# Autodesk Inventor assembly: 回転軸フレーム
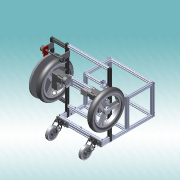
[picture p0: Inventor's stored thumbnail of the model, 180x180]
Saved by Autodesk Inventor 2015 (Build 190159000, 159)
## iProperties
Created: 2016-02-29
Part Number: 回転軸フレーム
Document SubType Name: Assembly
Designer: buzztaka
Author: buzztaka
## Documents named in this file (47)
- C:\Users\buzztaka\Downloads\2kk\i cart middle (main)  - コピー - コピー.iam
- C:\Users\buzztaka\Downloads\2kk\wheel_12inch.ipt
- C:\Users\buzztaka\Downloads\2kk\motor shaft.ipt
- C:\Users\buzztaka\Downloads\2kk\machine key L1.ipt
- C:\Users\buzztaka\Downloads\2kk\machine key L2.ipt
- C:\Users\buzztaka\Downloads\2kk\motor part2.ipt
- C:\Users\buzztaka\Downloads\2kk\wheel-cap.ipt
- C:\Users\buzztaka\Downloads\2kk\kw\wheel-hub.ipt
- C:\Users\buzztaka\Downloads\2kk\caster.ipt
- C:\Users\buzztaka\Downloads\2kk\motor fix plate.ipt
- C:\Users\buzztaka\Downloads\2kk\spacer for caster.ipt
- C:\Users\buzztaka\Downloads\2kk\motor part1.ipt
- C:\Users\buzztaka\Downloads\2kk\Aluminum Extrusions2020-L2.ipt
- C:\Users\buzztaka\Downloads\2kk\Aluminum Extrusions2040-L2.ipt
- C:\Users\buzztaka\Downloads\2kk\Aluminum Extrusions2060-L2.ipt
- C:\Users\buzztaka\Downloads\2kk\Aluminum Extrusions2040-L3.ipt
- C:\Users\buzztaka\Downloads\2kk\Aluminum Extrusions2020-L4.ipt
- C:\Users\buzztaka\Downloads\2kk\Aluminum Extrusions2020-L5.ipt
- C:\Users\buzztaka\Downloads\2kk\Aluminum Extrusions2020-L6.ipt
- C:\Users\buzztaka\Downloads\2kk\Aluminum Extrusions2020-L7.ipt
- C:\Users\buzztaka\Downloads\2kk\hblfsn5.ipt
- C:\Users\buzztaka\Downloads\2kk\hblfsnf5.ipt
- C:\Users\buzztaka\Downloads\2kk\HBLFSSW5.ipt
- C:\Users\buzztaka\Downloads\2kk\hntaj5_5.ipt
- C:\Users\buzztaka\Downloads\2kk\Nat for Aluminum flame.ipt
- C:\Users\buzztaka\Downloads\2kk\Blind Joint Parts - Screw Joints.ipt
- C:\Users\buzztaka\Downloads\2kk\MTi-30.ipt
- C:\Users\buzztaka\Downloads\2kk\M5 washer.ipt
- C:\Users\buzztaka\Downloads\2kk\CapboltM5-10.ipt
- C:\Users\buzztaka\Downloads\2kk\CapboltM5-8.ipt
- C:\Users\buzztaka\Downloads\2kk\spring washer M5.ipt
- C:\Users\buzztaka\Downloads\2kk\spring washer M3.ipt
- C:\Users\buzztaka\Downloads\2kk\Capbolt-M3-6.ipt
- C:\Users\buzztaka\Downloads\2kk\CapboltM5-60.ipt
- C:\Users\buzztaka\Downloads\2kk\CapboltM6-10.ipt
- C:\Users\buzztaka\Downloads\2kk\M3ネジ16mm.ipt
- C:\Users\buzztaka\Downloads\2kk\washer M5.ipt
- C:\Users\buzztaka\Downloads\2kk\kw\HFSB5-2020-550-LCH-RWV-AH30-BH240-CH280-DH442-EH462.ipt
- C:\Users\buzztaka\Downloads\2kk\kw\HFSB5-2020-550-LCH-RWV-AH30-BH60-CH85-DH240-EH280-AP442.ipt
- C:\Users\buzztaka\Downloads\2kk\kw\C-SFL6901ZZ.ipt
- C:\Users\buzztaka\Downloads\2kk\kw\HFSB5-2020-432-LCH-RCH-AH40-BH65 - (板用溝有り).ipt
- C:\Users\buzztaka\Downloads\2kk\回転軸取り付け板.ipt
- C:\Users\buzztaka\Downloads\2kk\計測輪周り - コピー.iam
- C:\Users\buzztaka\Downloads\2kk\HFSB5-2020-110-TPW .ipt
- C:\Users\buzztaka\Downloads\2kk\WSSS16-12-(ワッシャ12mm).ipt
- C:\Users\buzztaka\Downloads\2kk\シャフトホルダ12mm\SSTHMR12b.ipt
- C:\Users\buzztaka\Downloads\2kk\回転軸\SSFHR12-185.iam
## Components (255 placed, 46 different names)
1. wheel_12inch
2. motor shaft:1
3. machine key L1:1
4. machine key L2:1
5. motor part2:1
6. wheel-cap
7. wheel-hub
8. caster:1
9. motor fix plate:1
10. motor fix plate:2
11. spacer for caster:1
12. motor part1:1
13. spacer for caster:2
14. Aluminum Extrusions2020-L2:1
15. Aluminum Extrusions2040-L2:1
16. Aluminum Extrusions2060-L2:1 — 挿入:3, 挿入:4
17. Aluminum Extrusions2020-L2:2
18. Aluminum Extrusions2020-L2:3
19. Aluminum Extrusions2020-L2:4
20. Aluminum Extrusions2020-L2:5
21. Aluminum Extrusions2020-L2:6
22. Aluminum Extrusions2040-L3:1
23. Aluminum Extrusions2020-L4:1
24. Aluminum Extrusions2020-L5:1
25. Aluminum Extrusions2020-L6:1
26. Aluminum Extrusions2020-L7:1
27. hblfsn5
28. hblfsnf5:1
29. hblfsnf5:2
30. HBLFSSW5
31. hntaj5_5:1
32. hntaj5_5:2
33. Nat for Aluminum flame:1
34. Nat for Aluminum flame:2
35. Nat for Aluminum flame:3
36. Nat for Aluminum flame:4
37. hntaj5_5:3
38. hntaj5_5:4
39. hntaj5_5:5
40. hntaj5_5:6
41. hntaj5_5:12
42. Nat for Aluminum flame:5
43. Blind Joint Parts - Screw Joints:1
44. Blind Joint Parts - Screw Joints:2
45. Blind Joint Parts - Screw Joints:3
46. Blind Joint Parts - Screw Joints:4
47. Blind Joint Parts - Screw Joints:5
48. Blind Joint Parts - Screw Joints:6
49. Blind Joint Parts - Screw Joints:7
50. Blind Joint Parts - Screw Joints:8
51. Blind Joint Parts - Screw Joints:9
52. Blind Joint Parts - Screw Joints:10
53. Nat for Aluminum flame:6
54. Nat for Aluminum flame:7
55. Nat for Aluminum flame:8
56. Nat for Aluminum flame:9
57. Nat for Aluminum flame:10
58. Nat for Aluminum flame:11
59. Nat for Aluminum flame:12
60. Nat for Aluminum flame:13
61. Nat for Aluminum flame:14
62. hntaj5_5:16
63. hntaj5_5:17
64. hntaj5_5:18
65. hntaj5_5:19
66. hntaj5_5:20
67. hntaj5_5:21
68. hntaj5_5:22
69. hntaj5_5:23
70. Blind Joint Parts - Screw Joints:11
71. Blind Joint Parts - Screw Joints:12
72. hntaj5_5:24
73. hntaj5_5:25
74. caster:2
75. Aluminum Extrusions2040-L3:2
76. wheel_12inch:1
77. motor fix plate:3
78. motor fix plate:4
79. wheel-cap:1
80. machine key L2:2
81. motor shaft:2
82. machine key L1:2
83. wheel-hub:1
84. MTi-30
85. Aluminum Extrusions2020-L4:2
86. Aluminum Extrusions2020-L5:2
87. hblfsn5:1
88. Aluminum Extrusions2020-L6:2
89. Aluminum Extrusions2020-L7:2
90. CapboltM5-10:2
91. CapboltM5-10:3
92. CapboltM5-10:4
93. CapboltM5-10:5
94. CapboltM5-8:1
95. CapboltM5-8:2
96. CapboltM5-10:6
97. CapboltM5-10:7
98. CapboltM5-10:8
99. CapboltM5-10:9
100. CapboltM5-10:12
101. CapboltM5-10:13
102. CapboltM5-8:6
103. CapboltM5-8:7
104. CapboltM5-8:8
105. CapboltM5-10:14
106. CapboltM5-10:15
107. CapboltM5-10:16
108. CapboltM5-10:17
109. CapboltM5-10:18
110. CapboltM5-10:19
111. CapboltM5-8:12
112. spring washer M5:4
113. CapboltM5-8:13
114. spring washer M5:5
115. Capbolt-M3-6:3
116. spring washer M3:3
117. CapboltM5-60:1
118. CapboltM6-10:1
119. M3ネジ16mm:1
120. washer M5:1
121. spring washer M5:6
122. M5 washer:2
123. washer M5:2
124. spring washer M5:7 — 挿入:47
125. CapboltM5-8:15
126. spring washer M5:8
127. M5 washer:3
128. CapboltM5-60:2
129. spring washer M5:9
130. CapboltM5-10:20
131. CapboltM5-8:16
132. spring washer M5:10
133. CapboltM5-8:17
134. spring washer M5:11
135. CapboltM5-8:18
136. spring washer M5:12
137. CapboltM5-8:19
138. spring washer M5:13
139. CapboltM5-8:20
140. spring washer M5:14
141. CapboltM5-8:21
142. spring washer M5:15
143. hblfsnf5:3
144. Blind Joint Parts - Screw Joints:16
145. Blind Joint Parts - Screw Joints:17
146. Blind Joint Parts - Screw Joints:18
147. Blind Joint Parts - Screw Joints:19
148. hntaj5_5:26
149. CapboltM5-10:21
150. CapboltM5-10:22
151. Nat for Aluminum flame:15
152. Blind Joint Parts - Screw Joints:20
153. Blind Joint Parts - Screw Joints:21
154. Nat for Aluminum flame:16
155. CapboltM5-8:22
156. Nat for Aluminum flame:17
157. CapboltM5-8:23
158. hntaj5_5:27
159. CapboltM5-10:23
160. hntaj5_5:28
161. CapboltM5-10:24
162. Blind Joint Parts - Screw Joints:22
163. Blind Joint Parts - Screw Joints:23
164. Blind Joint Parts - Screw Joints:24
165. Blind Joint Parts - Screw Joints:25
166. Nat for Aluminum flame:18
167. CapboltM5-10:27
168. CapboltM5-10:28
169. Nat for Aluminum flame:19
170. Nat for Aluminum flame:20
171. CapboltM5-10:29
172. Nat for Aluminum flame:21
173. CapboltM5-10:30
174. Nat for Aluminum flame:22
175. CapboltM5-10:31
176. CapboltM5-10:32
177. Nat for Aluminum flame:23
178. spring washer M3:13
179. spring washer M3:14
180. Capbolt-M3-6:13
181. Capbolt-M3-6:14
182. CapboltM6-10:2
183. CapboltM6-10:3
184. CapboltM6-10:4
185. CapboltM5-10:33
186. CapboltM5-10:34
187. CapboltM5-10:35
188. CapboltM5-10:36
189. CapboltM5-10:37
190. CapboltM6-10:5
191. CapboltM6-10:6
192. CapboltM6-10:7
193. CapboltM6-10:8
194. CapboltM5-10:38
195. CapboltM5-10:39
196. M3ネジ16mm:2
197. M3ネジ16mm:3
198. M3ネジ16mm:4
199. hntaj5_5:35
200. Blind Joint Parts - Screw Joints:26
201. CapboltM5-8:28
202. spring washer M5:17
203. CapboltM5-8:29
204. spring washer M5:18
205. hntaj5_5:36
206. CapboltM5-8:30
207. spring washer M5:19
208. hntaj5_5:37
209. hntaj5_5:38
210. CapboltM5-8:31
211. spring washer M5:20
212. washer M5:3
213. CapboltM5-8:32
214. spring washer M5:21
215. M3ネジ16mm:5
216. M3ネジ16mm:6
217. M3ネジ16mm:7
218. CapboltM5-60:3
219. spring washer M5:22
220. M3ネジ16mm:8
221. spring washer M5:23
222. CapboltM5-60:4
223. CapboltM5-8:33
224. washer M5:4
225. M5 washer:4
226. M5 washer:5
227. hntaj5_5:39
228. CapboltM5-8:34
229. spring washer M5:24
230. CapboltM5-8:35
231. spring washer M5:25
232. hntaj5_5:40
233. CapboltM5-8:36
234. spring washer M5:26
235. hntaj5_5:42
236. hntaj5_5:42
237. spring washer M5:27
238. CapboltM5-8:37
239. spring washer M5:28
240. HFSB5-2020-550-LCH-RWV-AH30-BH240-CH280-DH442-EH462:2 — 挿入:3, 挿入:4
241. HFSB5-2020-550-LCH-RWV-AH30-BH60-CH85-DH240-EH280-AP442:1 — 挿入:32, 挿入:33, 挿入:39, 挿入:40
242. C-SFL6901ZZ:2 — 挿入:54, 挿入:56
243. 回転軸取り付け板:1 — 挿入:32, 挿入:33, 挿入:56
244. HFSB5-2020-110-TPW :1 — 挿入:39, 挿入:42
245. HFSB5-2020-110-TPW :2 — 挿入:40, 挿入:41
246. 計測輪周り - コピー:1 [sub-assembly] — 挿入:46
247. HFSB5-2020-432-LCH-RCH-AH40-BH65 - (板用溝有り):2 — 挿入:41, 挿入:42, 挿入:43, 挿入:44
248. C-SFL6901ZZ:3 — 挿入:45, 挿入:46, 挿入:52
249. 回転軸取り付け板:2 — 挿入:43, 挿入:44, 挿入:45
250. CapboltM5-8:38 — 挿入:47
251. WSSS16-12-(ワッシャ12mm):1 — 挿入:52, 挿入:53
252. SSTHMR12b:1 — 挿入:53, 挿入:57
253. SSTHMR12b:2 — 挿入:55
254. WSSS16-12-(ワッシャ12mm):2 — 挿入:54, 挿入:55
255. SSFHR12-185:1 [sub-assembly] — 挿入:57
## Relationships (21: Insert 21)
- 挿入:3 [Insert]: Aluminum Extrusions2060-L2:1 ↔ HFSB5-2020-550-LCH-RWV-AH30-BH240-CH280-DH442-EH462:2
- 挿入:4 [Insert]: Aluminum Extrusions2060-L2:1 ↔ HFSB5-2020-550-LCH-RWV-AH30-BH240-CH280-DH442-EH462:2
- [Insert]: Aluminum Extrusions2020-L2:1 ↔ HFSB5-2020-550-LCH-RWV-AH30-BH60-CH85-DH240-EH280-AP442:1
- [Insert]: Aluminum Extrusions2060-L2:1 ↔ HFSB5-2020-550-LCH-RWV-AH30-BH60-CH85-DH240-EH280-AP442:1
- 挿入:32 [Insert]: HFSB5-2020-550-LCH-RWV-AH30-BH60-CH85-DH240-EH280-AP442:1 ↔ 回転軸取り付け板:1
- 挿入:33 [Insert]: HFSB5-2020-550-LCH-RWV-AH30-BH60-CH85-DH240-EH280-AP442:1 ↔ 回転軸取り付け板:1
- 挿入:39 [Insert]: HFSB5-2020-550-LCH-RWV-AH30-BH60-CH85-DH240-EH280-AP442:1 ↔ HFSB5-2020-110-TPW :1
- 挿入:40 [Insert]: HFSB5-2020-550-LCH-RWV-AH30-BH60-CH85-DH240-EH280-AP442:1 ↔ HFSB5-2020-110-TPW :2
- 挿入:41 [Insert]: HFSB5-2020-110-TPW :2 ↔ HFSB5-2020-432-LCH-RCH-AH40-BH65 - (板用溝有り):2
- 挿入:42 [Insert]: HFSB5-2020-110-TPW :1 ↔ HFSB5-2020-432-LCH-RCH-AH40-BH65 - (板用溝有り):2
- 挿入:43 [Insert]: HFSB5-2020-432-LCH-RCH-AH40-BH65 - (板用溝有り):2 ↔ 回転軸取り付け板:2
- 挿入:44 [Insert]: HFSB5-2020-432-LCH-RCH-AH40-BH65 - (板用溝有り):2 ↔ 回転軸取り付け板:2
- 挿入:45 [Insert]: C-SFL6901ZZ:3 ↔ 回転軸取り付け板:2
- 挿入:46 [Insert]: 計測輪周り - コピー:1 ↔ C-SFL6901ZZ:3
- 挿入:47 [Insert]: spring washer M5:7 ↔ CapboltM5-8:38
- 挿入:52 [Insert]: C-SFL6901ZZ:3 ↔ WSSS16-12-(ワッシャ12mm):1
- 挿入:53 [Insert]: WSSS16-12-(ワッシャ12mm):1 ↔ SSTHMR12b:1
- 挿入:54 [Insert]: C-SFL6901ZZ:2 ↔ WSSS16-12-(ワッシャ12mm):2
- 挿入:55 [Insert]: SSTHMR12b:2 ↔ WSSS16-12-(ワッシャ12mm):2
- 挿入:56 [Insert]: C-SFL6901ZZ:2 ↔ 回転軸取り付け板:1
- 挿入:57 [Insert]: SSTHMR12b:1 ↔ SSFHR12-185:1
